# Autodesk Inventor assembly: Whole_Assembly
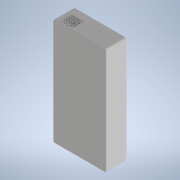
[picture p0: Inventor's stored thumbnail of the model, 180x180]
Saved by Autodesk Inventor 2021 (Build 250183000, 183)
## iProperties
Created: 2020-07-29
Part Number: Whole_Assembly
Document SubType Name: Assembly
Designer: ridvansong
Author: ridvansong
## Documents named in this file (4)
- \\Mac\Home\Documents\OP-1 Project\ipt_files\Whole_Assembly.iam
- \\Mac\Home\Documents\OP-1 Project\ipt_files\Backboard.ipt
- \\Mac\Home\Documents\OP-1 Project\ipt_files\Base.ipt
- \\Mac\Home\Documents\OP-1 Project\ipt_files\Cover.ipt
## Components (3 placed, 3 different names)
1. Backboard:1 — Mate:1, Mate:3, Mate:4
2. Base:1 — Mate:1, Flush:1, Flush:2, Mate:2, Mate:3, Mate:4
3. Cover:1 — Flush:1, Flush:2, Mate:2
## Relationships (6: Mate 4, Flush 2)
- Mate:1: Backboard:1 ↔ Base:1
- Flush:1: Base:1 ↔ Cover:1
- Flush:2: Base:1 ↔ Cover:1
- Mate:2: Base:1 ↔ Cover:1
- Mate:3 (3 mm): Backboard:1 ↔ Base:1
- Mate:4 (3 mm): Backboard:1 ↔ Base:1
